# Autodesk Inventor assembly: 000.000 - Короб электроники
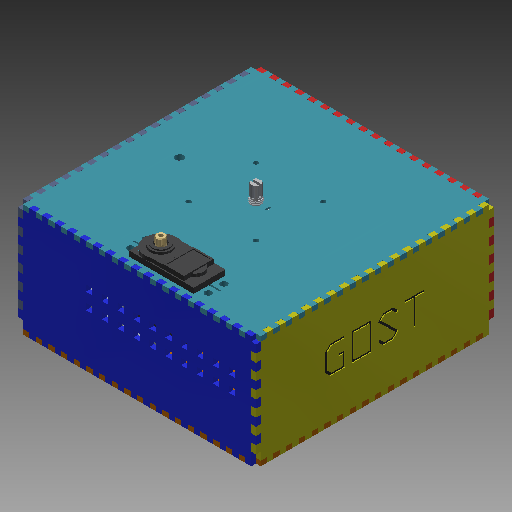
[picture p0: Inventor's stored thumbnail of the model, 512x512]
Saved by Autodesk Inventor 2019 (Build 230136000, 136)
## iProperties
Created: 2020-02-27
Part Number: 000.000 - Короб электроники
Material: Типовые
Document SubType Name: Assembly
Designer: Петров Иван
Author: Петров Иван
## Documents named in this file (13)
- E:\IVAN\Ivan_desktop\GitHub\Manipulation_IRS\hardware\5-DOF\000.200 - Короб электроники.iam
- E:\IVAN\Ivan_desktop\GitHub\Manipulation_IRS\hardware\5-DOF\000.201 - Дно.ipt
- E:\IVAN\Ivan_desktop\GitHub\Manipulation_IRS\hardware\5-DOF\000.202 - Боковая стенка пустая.ipt
- E:\IVAN\Ivan_desktop\GitHub\Manipulation_IRS\hardware\5-DOF\000.203 - Боковая стенка лицевая.ipt
- E:\IVAN\Ivan_desktop\GitHub\Manipulation_IRS\hardware\5-DOF\000.204 - Боковая стенка управляющая.ipt
- E:\IVAN\Ivan_desktop\GitHub\Manipulation_IRS\hardware\5-DOF\000.205 - Боковая стенка винтелиационная.ipt
- E:\IVAN\Ivan_desktop\GitHub\Manipulation_IRS\hardware\5-DOF\000.206 - Крышка.ipt
- E:\IVAN\Ivan_desktop\GitHub\Manipulation_IRS\hardware\5-DOF\components\tower prone.ipt
- E:\IVAN\Ivan_desktop\GitHub\Manipulation_IRS\hardware\5-DOF\components\Potentiometer.ipt
- E:\IVAN\Ivan_desktop\GitHub\Manipulation_IRS\hardware\5-DOF\000.207 - Поддержка центра.ipt
- E:\IVAN\Ivan_desktop\GitHub\Manipulation_IRS\hardware\5-DOF\components\Raspberry Pi 3.ipt
- E:\IVAN\Ivan_desktop\GitHub\Manipulation_IRS\hardware\5-DOF\components\NUCLEO.ipt
- E:\IVAN\Ivan_desktop\GitHub\Manipulation_IRS\hardware\5-DOF\components\tattu 1300MHa 3s LiPo.ipt
## Components (12 placed, 12 different names)
1. 000.201 - Дно:1 — Заподлицо:1, Совмещение:1, Совмещение:2, Совмещение:3, Совмещение:4, Совмещение:5, Совмещение:6, Совмещение:7, Совмещение:8, Совмещение:24, Совмещение:31, Совмещение:32, Совмещение:33, Совмещение:36, Совмещение:38, Совмещение:39, Совмещение:41
2. 000.202 - Боковая стенка пустая:1 — Заподлицо:1, Совмещение:1, Совмещение:2, Заподлицо:5
3. 000.203 - Боковая стенка лицевая:1 — Совмещение:3, Совмещение:4, Совмещение:5, Заподлицо:2, Совмещение:9, Заподлицо:3, Совмещение:10
4. 000.204 - Боковая стенка управляющая:1 — Совмещение:6, Совмещение:7, Заподлицо:2, Совмещение:40, Совмещение:42, Заподлицо:4
5. 000.205 - Боковая стенка винтелиационная:1 — Совмещение:8, Совмещение:9, Заподлицо:3
6. 000.206 - Крышка:1 — Совмещение:10, Совмещение:11, Совмещение:12, Совмещение:13, Совмещение:18, Совмещение:19, Совмещение:20, Заподлицо:4, Заподлицо:5
7. tower prone:1 — Совмещение:11, Совмещение:12, Совмещение:13
8. Potentiometer:1 — Совмещение:18, Совмещение:19, Совмещение:20
9. 000.207 - Поддержка центра:1 — Совмещение:24, Совмещение:32, Совмещение:33
10. Raspberry Pi 3:1 — Совмещение:31, Совмещение:38, Совмещение:39
11. NUCLEO:1 — Совмещение:36, Совмещение:40
12. tattu 1300MHa 3s LiPo:1 — Совмещение:41, Совмещение:42
## Relationships (31: Mate 26, Flush 5)
- Заподлицо:1 [Flush]: 000.201 - Дно:1 ↔ 000.202 - Боковая стенка пустая:1
- Совмещение:1 [Mate]: 000.201 - Дно:1 ↔ 000.202 - Боковая стенка пустая:1
- Совмещение:2 [Mate]: 000.201 - Дно:1 ↔ 000.202 - Боковая стенка пустая:1
- Совмещение:3 [Mate]: 000.201 - Дно:1 ↔ 000.203 - Боковая стенка лицевая:1
- Совмещение:4 [Mate]: 000.201 - Дно:1 ↔ 000.203 - Боковая стенка лицевая:1
- Совмещение:5 [Mate]: 000.201 - Дно:1 ↔ 000.203 - Боковая стенка лицевая:1
- Совмещение:6 [Mate]: 000.201 - Дно:1 ↔ 000.204 - Боковая стенка управляющая:1
- Совмещение:7 [Mate]: 000.201 - Дно:1 ↔ 000.204 - Боковая стенка управляющая:1
- Заподлицо:2 [Flush]: 000.203 - Боковая стенка лицевая:1 ↔ 000.204 - Боковая стенка управляющая:1
- Совмещение:8 [Mate]: 000.201 - Дно:1 ↔ 000.205 - Боковая стенка винтелиационная:1
- Совмещение:9 [Mate]: 000.203 - Боковая стенка лицевая:1 ↔ 000.205 - Боковая стенка винтелиационная:1
- Заподлицо:3 [Flush]: 000.203 - Боковая стенка лицевая:1 ↔ 000.205 - Боковая стенка винтелиационная:1
- Совмещение:10 [Mate]: 000.203 - Боковая стенка лицевая:1 ↔ 000.206 - Крышка:1
- Совмещение:11 [Mate]: 000.206 - Крышка:1 ↔ tower prone:1
- Совмещение:12 [Mate]: 000.206 - Крышка:1 ↔ tower prone:1
- Совмещение:13 [Mate]: 000.206 - Крышка:1 ↔ tower prone:1
- Совмещение:18 [Mate]: 000.206 - Крышка:1 ↔ Potentiometer:1
- Совмещение:19 [Mate]: 000.206 - Крышка:1 ↔ Potentiometer:1
- Совмещение:20 [Mate]: 000.206 - Крышка:1 ↔ Potentiometer:1
- Совмещение:24 [Mate]: 000.201 - Дно:1 ↔ 000.207 - Поддержка центра:1
- Совмещение:31 [Mate] (5 mm): 000.201 - Дно:1 ↔ Raspberry Pi 3:1
- Совмещение:32 [Mate]: 000.201 - Дно:1 ↔ 000.207 - Поддержка центра:1
- Совмещение:33 [Mate]: 000.201 - Дно:1 ↔ 000.207 - Поддержка центра:1
- Совмещение:36 [Mate] (15 mm): 000.201 - Дно:1 ↔ NUCLEO:1
- Совмещение:38 [Mate]: 000.201 - Дно:1 ↔ Raspberry Pi 3:1
- Совмещение:39 [Mate]: 000.201 - Дно:1 ↔ Raspberry Pi 3:1
- Совмещение:40 [Mate] (2 mm): 000.204 - Боковая стенка управляющая:1 ↔ NUCLEO:1
- Совмещение:41 [Mate]: 000.201 - Дно:1 ↔ tattu 1300MHa 3s LiPo:1
- Совмещение:42 [Mate] (8 mm): 000.204 - Боковая стенка управляющая:1 ↔ tattu 1300MHa 3s LiPo:1
- Заподлицо:4 [Flush]: 000.204 - Боковая стенка управляющая:1 ↔ 000.206 - Крышка:1
- Заподлицо:5 [Flush]: 000.202 - Боковая стенка пустая:1 ↔ 000.206 - Крышка:1
